# Autodesk Inventor assembly: chaimber-bolt
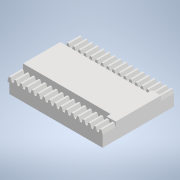
[picture p0: Inventor's stored thumbnail of the model, 180x180]
Saved by Autodesk Inventor 2021 (Build 250183000, 183)
## iProperties
Created: 2024-03-18
Part Number: chaimber-bolt
Document SubType Name: Assembly
Designer: 22hamfri
Author: 22hamfri
## Documents named in this file (3)
- C:\Users\22hamfri\Documents\School\Programmering\domino-bil\CAD\chaimber-bolt.iam
- C:\Users\22hamfri\Documents\School\Programmering\domino-bil\CAD\chaimber-bolt.ipt
- C:\Users\22hamfri\Documents\School\Programmering\domino-bil\CAD\bolt-rack.ipt
## Components (3 placed, 2 different names)
1. chaimber-bolt:1 — Rigid:1, Rigid:2
2. bolt-rack:1 — Rigid:1
3. bolt-rack:2 — Rigid:2
## Relationships (2: WeldJoint 2)
- Rigid:1 [WeldJoint]: chaimber-bolt:1 ↔ bolt-rack:1
- Rigid:2 [WeldJoint]: chaimber-bolt:1 ↔ bolt-rack:2
